# Autodesk Inventor assembly: 00_Linear_rail_Y
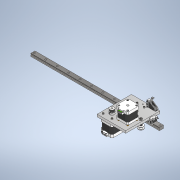
[picture p0: Inventor's stored thumbnail of the model, 180x180]
Saved by Autodesk Inventor 2022.2 (Build 262287010, 287A)
## iProperties
Created: 2022-05-03
Part Number: 00_Linear_rail_Y
Document SubType Name: Assembly
Designer: MXBD
Author: MXBD
## Documents named in this file (8)
- D:\Laser_Engraver\CAD\Assembly\00_Linear_rail_Y.iam
- D:\Laser_Engraver\CAD\Parts\02_mgn15h_Rail_450mm.ipt
- D:\Laser_Engraver\CAD\Parts\01_mgn15h_Bearing_Block.ipt
- D:\Laser_Engraver\CAD\Assembly\02_Baseplate.iam
- C:\Users\49152\Documents\Inventor\Content Center Files\R2022\de-DE\ISO 4762(2)\ISO 4762 - M3 x 12ISO.ipt
- D:\Laser_Engraver\CAD\Parts\06_Micro_Limit_Switch.ipt
- D:\Laser_Engraver\CAD\Parts\27_Switch_Holder_X.ipt
- D:\Laser_Engraver\CAD\Parts\28_Switch_Holder_Y.ipt
## Components (11 placed, 7 different names)
1. 02_mgn15h_Rail_450mm:1 — Passend:1, Passend:2, Passend:17, Passend:18, Winkel:1
2. 01_mgn15h_Bearing_Block:1 — Passend:1, Passend:2, Passend:3, Passend:4, Passend:5
3. 02_Baseplate:1 [sub-assembly] — Passend:3, Passend:4, Passend:5, Passend:6, Passend:7, Passend:8, Passend:9, Passend:10, Passend:11, Passend:12, Passend:13, Passend:14, Fluchtend:1, Fluchtend:2, Passend:15, Fluchtend:3
4. ISO 4762 M3 x 12:1 — Passend:6, Passend:13
5. ISO 4762 M3 x 12:2 — Passend:7, Passend:12
6. ISO 4762 M3 x 12:3 — Passend:8, Passend:10
7. ISO 4762 M3 x 12:4 — Passend:9, Passend:11
8. 06_Micro_Limit_Switch:1 — Passend:14, Fluchtend:1, Fluchtend:2, Passend:16
9. 27_Switch_Holder_X:1 — Passend:15, Passend:16, Fluchtend:3
10. 28_Switch_Holder_Y:1 — Passend:17, Passend:18, Fluchtend:4, Fluchtend:5, Passend:19, Winkel:1
11. 06_Micro_Limit_Switch:2 — Fluchtend:4, Fluchtend:5, Passend:19
## Relationships (25: Mate 19, Flush 5, Angle 1)
- Passend:1 [Mate]: 02_mgn15h_Rail_450mm:1 ↔ 01_mgn15h_Bearing_Block:1
- Passend:2 [Mate]: 02_mgn15h_Rail_450mm:1 ↔ 01_mgn15h_Bearing_Block:1
- Passend:3 [Mate]: 01_mgn15h_Bearing_Block:1 ↔ 02_Baseplate:1
- Passend:4 [Mate]: 01_mgn15h_Bearing_Block:1 ↔ 02_Baseplate:1
- Passend:5 [Mate]: 01_mgn15h_Bearing_Block:1 ↔ 02_Baseplate:1
- Passend:6 [Mate]: 02_Baseplate:1 ↔ ISO 4762 M3 x 12:1
- Passend:7 [Mate]: 02_Baseplate:1 ↔ ISO 4762 M3 x 12:2
- Passend:8 [Mate]: 02_Baseplate:1 ↔ ISO 4762 M3 x 12:3
- Passend:9 [Mate]: 02_Baseplate:1 ↔ ISO 4762 M3 x 12:4
- Passend:10 [Mate]: 02_Baseplate:1 ↔ ISO 4762 M3 x 12:3
- Passend:11 [Mate]: 02_Baseplate:1 ↔ ISO 4762 M3 x 12:4
- Passend:12 [Mate]: 02_Baseplate:1 ↔ ISO 4762 M3 x 12:2
- Passend:13 [Mate]: 02_Baseplate:1 ↔ ISO 4762 M3 x 12:1
- Passend:14 [Mate]: 02_Baseplate:1 ↔ 06_Micro_Limit_Switch:1
- Fluchtend:1 [Flush]: 02_Baseplate:1 ↔ 06_Micro_Limit_Switch:1
- Fluchtend:2 [Flush] (30 mm): 02_Baseplate:1 ↔ 06_Micro_Limit_Switch:1
- Passend:15 [Mate]: 02_Baseplate:1 ↔ 27_Switch_Holder_X:1
- Passend:16 [Mate]: 06_Micro_Limit_Switch:1 ↔ 27_Switch_Holder_X:1
- Fluchtend:3 [Flush]: 02_Baseplate:1 ↔ 27_Switch_Holder_X:1
- Passend:17 [Mate]: 02_mgn15h_Rail_450mm:1 ↔ 28_Switch_Holder_Y:1
- Passend:18 [Mate]: 02_mgn15h_Rail_450mm:1 ↔ 28_Switch_Holder_Y:1
- Fluchtend:4 [Flush]: 28_Switch_Holder_Y:1 ↔ 06_Micro_Limit_Switch:2
- Fluchtend:5 [Flush]: 28_Switch_Holder_Y:1 ↔ 06_Micro_Limit_Switch:2
- Passend:19 [Mate]: 28_Switch_Holder_Y:1 ↔ 06_Micro_Limit_Switch:2
- Winkel:1 [Angle] (0 deg): 02_mgn15h_Rail_450mm:1 ↔ 28_Switch_Holder_Y:1
